# Autodesk Inventor assembly: Ensamblaje Reloj LCD 16x2
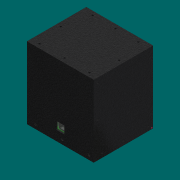
[picture p0: Inventor's stored thumbnail of the model, 180x180]
Saved by Autodesk Inventor 2019 (Build 230136000, 136)
## iProperties
Created: 2024-12-30
Part Number: Ensamblaje Reloj LCD 16x2
Document SubType Name: Assembly
Designer: Familia CS
Author: Familia CS
## Documents named in this file (10)
- G:\Mi unidad\Mis Proyectos\Reloj Digital LCD 16 x 2\Inventor\Caja de reloj 16x2 LCD\Caja esamblaje\Ensamblaje Reloj LCD 16x2.iam
- G:\Mi unidad\Mis Proyectos\Reloj Digital LCD 16 x 2\Inventor\Caja de reloj 16x2 LCD\Caja esamblaje\3D\PCB Down.ipt
- G:\Mi unidad\Mis Proyectos\Reloj Digital LCD 16 x 2\Inventor\Caja de reloj 16x2 LCD\Caja esamblaje\Lado Down\Down.ipt
- G:\Mi unidad\Mis Proyectos\Reloj Digital LCD 16 x 2\Inventor\Caja de reloj 16x2 LCD\Caja esamblaje\Lado Before\Before.ipt
- G:\Mi unidad\Mis Proyectos\Reloj Digital LCD 16 x 2\Inventor\Caja de reloj 16x2 LCD\Caja esamblaje\Lateral Derecho\Lateral Derecho.ipt
- G:\Mi unidad\Mis Proyectos\Reloj Digital LCD 16 x 2\Inventor\Caja de reloj 16x2 LCD\Caja esamblaje\Lateral Izquierdo\3D\Lado izquierdo.ipt
- G:\Mi unidad\Mis Proyectos\Reloj Digital LCD 16 x 2\Inventor\Caja de reloj 16x2 LCD\Caja esamblaje\Lado UP\3D\UP.ipt
- G:\Mi unidad\Mis Proyectos\Reloj Digital LCD 16 x 2\Inventor\Caja de reloj 16x2 LCD\Caja esamblaje\Lado Front\3D\Front.ipt
- G:\Mi unidad\Mis Proyectos\Reloj Digital LCD 16 x 2\Inventor\Separadores\3D\PCB SEPARADOR.ipt
- G:\Mi unidad\Mis Proyectos\Reloj Digital LCD 16 x 2\Inventor\Caja de reloj 16x2 LCD\Caja esamblaje\3D\PCB Front.ipt
## Components (12 placed, 9 different names)
1. PCB Down:1 — Flush:1, Flush:2
2. Down:1 — Flush:1, Flush:2, Flush:3, Flush:4, Flush:5, Flush:6, Flush:7, Flush:8, Flush:11, Flush:12
3. Before:1 — Flush:3, Flush:4, Flush:9, Flush:10
4. Lateral Derecho:1 — Flush:5, Flush:6
5. Lado izquierdo:1 — Flush:7, Flush:8
6. UP:1 — Flush:9, Flush:10, Flush:13
7. Front:1 — Flush:11, Flush:12, Flush:13, Rigid:1, Rotational:1, Rotational:2, Rotational:3
8. PCB SEPARADOR:1 — Rigid:1
9. PCB SEPARADOR:2 — Rotational:2
10. PCB SEPARADOR:3 — Rotational:3, Insert:1
11. PCB SEPARADOR:4 — Rotational:1
12. PCB Front:1 — Insert:1
## Relationships (18: Flush 13, RevoluteJoint 3, WeldJoint 1, Insert 1)
- Flush:1: PCB Down:1 ↔ Down:1
- Flush:2: PCB Down:1 ↔ Down:1
- Flush:3: Down:1 ↔ Before:1
- Flush:4: Down:1 ↔ Before:1
- Flush:5: Down:1 ↔ Lateral Derecho:1
- Flush:6: Down:1 ↔ Lateral Derecho:1
- Flush:7: Down:1 ↔ Lado izquierdo:1
- Flush:8: Down:1 ↔ Lado izquierdo:1
- Flush:9: Before:1 ↔ UP:1
- Flush:10: Before:1 ↔ UP:1
- Flush:11: Down:1 ↔ Front:1
- Flush:12: Down:1 ↔ Front:1
- Flush:13: UP:1 ↔ Front:1
- Rigid:1 [WeldJoint]: Front:1 ↔ PCB SEPARADOR:1
- Rotational:1 [RevoluteJoint]: Front:1 ↔ PCB SEPARADOR:4
- Rotational:2 [RevoluteJoint]: Front:1 ↔ PCB SEPARADOR:2
- Rotational:3 [RevoluteJoint]: Front:1 ↔ PCB SEPARADOR:3
- Insert:1: PCB SEPARADOR:3 ↔ PCB Front:1
